# Autodesk Inventor assembly: Gate_LED_Assembly
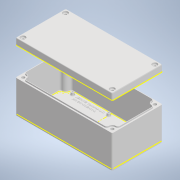
[picture p0: Inventor's stored thumbnail of the model, 180x180]
Saved by Autodesk Inventor 2021 (Build 250183000, 183)
## iProperties
Created: 2021-04-06
Part Number: Gate_LED_Assembly
Document SubType Name: Assembly
Designer: James
Author: James
## Documents named in this file (3)
- C:\Users\james\Dev\homeprojects\Electronics\XC-0001-Gate_LEDs Rev 3\3D Model\Gate_LED_Assembly.iam
- C:\Users\james\Dev\homeprojects\Electronics\XC-0001-Gate_LEDs Rev 3\3D Model\CustomBox_Rev3a.ipt
- C:\Users\james\Dev\homeprojects\Electronics\XC-0001-Gate_LEDs Rev 3\3D Model\CustomLid_Rev3a.ipt
## Components (2 placed, 2 different names)
1. CustomBox_Rev3a:1
2. CustomLid_Rev3a:1 — Flush:1
## Relationships (1: Flush 1)
- Flush:1: CustomLid_Rev3a:1
